# Autodesk Inventor assembly: V-Belt transmission
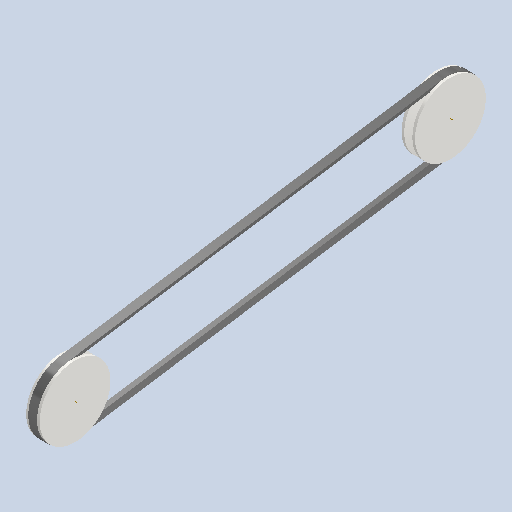
[picture p0: Inventor's stored thumbnail of the model, 512x512]
Saved by Autodesk Inventor 2024 (Build 280153000, 153)
## iProperties
ClientObjectVersion: 1
Created: 2024-05-11
Part Number: V-Belt transmission
Document SubType Name: Assembly
Designer: teeta
Author: teeta
## Documents named in this file (4)
- C:\Users\teeta\OneDrive\Documents\Inventor\Rophi'sProject\Assembly\Design Accelerator\V-Belt transmission5.iam
- C:\Users\teeta\OneDrive\Documents\Inventor\Rophi'sProject\Assembly\Design Accelerator\V-Belt5.ipt
- C:\Users\teeta\OneDrive\Documents\Inventor\Rophi'sProject\Assembly\Design Accelerator\Grooved Pulley15.ipt
- C:\Users\teeta\OneDrive\Documents\Inventor\Rophi'sProject\Assembly\Design Accelerator\Grooved Pulley25.ipt
## Components (3 placed, 3 different names)
1. Grooved Pulley1:1 — Flush:1, Mate:1, Rotation:1
2. Grooved Pulley2:1 — Flush:2, Mate:2, Rotation:1
3. V-Belt:1 — Flush:1, Mate:1, Flush:2, Mate:2
## Component patterns: (1 elements, first: V-Belt:1)
## Relationships (5: Flush 2, Mate 2, RelateRotation 1)
- Flush:1: Grooved Pulley1:1 ↔ V-Belt:1
- Mate:1: Grooved Pulley1:1 ↔ V-Belt:1
- Flush:2: Grooved Pulley2:1 ↔ V-Belt:1
- Mate:2: Grooved Pulley2:1 ↔ V-Belt:1
- Rotation:1 [RelateRotation] (1 ul): Grooved Pulley1:1 ↔ Grooved Pulley2:1
